# Autodesk Inventor assembly: SubAssembly
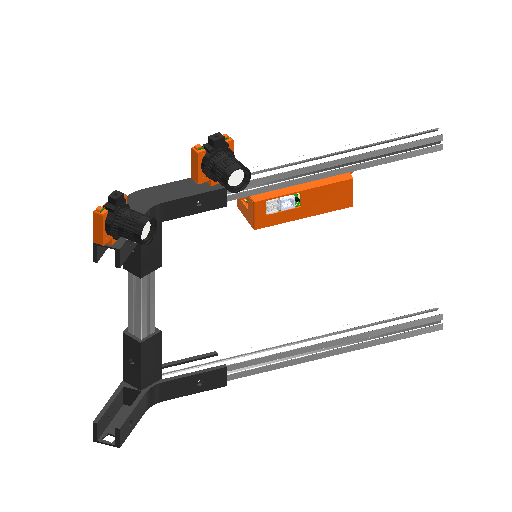
[picture p0: Inventor's stored thumbnail of the model, 512x512]
Saved by Autodesk Inventor 2025.2 (Build 292293000, 293)
## iProperties
Created: 2025-03-12
Part Number: SubAssembly
Document SubType Name: Assembly
Designer: rolan
Author: rolan
## Documents named in this file (6)
- C:\Users\rolan\Documents\PhD\Inventor\Assembly\SubAssembly.iam
- C:\Users\rolan\Documents\PhD\Inventor\Parts\135FootUpdate.ipt
- C:\Users\rolan\Documents\PhD\Inventor\Parts\Strut.ipt
- C:\Users\rolan\Documents\PhD\Inventor\Parts\Strut_short.ipt
- C:\Users\rolan\Documents\PhD\Inventor\Assembly\Camera.iam
- C:\Users\rolan\Documents\PhD\Inventor\Assembly\StereoPi.iam
## Components (8 placed, 5 different names)
1. 135FootUpdate:1 — Mate:1, Mate:2, Mate:3, Mate:26
2. Strut:1 — Mate:1, Mate:2, Mate:3
3. 135FootUpdate:2 — Mate:10, Mate:11, Mate:12, Mate:14, Mate:15, Flush:1, Mate:16, Mate:17, Mate:20, Mate:21, Mate:22, Mate:23, Mate:24, Mate:25
4. Strut:2 — Mate:10, Mate:11, Mate:12, Mate:13, Mate:18, Flush:20
5. Camera:1 [sub-assembly] — Mate:13, Mate:14, Mate:15, Mate:22, Mate:23
6. Camera:2 [sub-assembly] — Flush:1, Mate:16, Mate:17, Mate:20, Mate:21
7. StereoPi:1 [sub-assembly] — Mate:18, Flush:20
8. Strut_short:1 — Mate:24, Mate:25, Mate:26
## Relationships (21: Mate 19, Flush 2)
- Mate:1: 135FootUpdate:1 ↔ Strut:1
- Mate:2: 135FootUpdate:1 ↔ Strut:1
- Mate:3: 135FootUpdate:1 ↔ Strut:1
- Mate:10: 135FootUpdate:2 ↔ Strut:2
- Mate:11: 135FootUpdate:2 ↔ Strut:2
- Mate:12: 135FootUpdate:2 ↔ Strut:2
- Mate:13: Strut:2 ↔ Camera:1
- Mate:14: 135FootUpdate:2 ↔ Camera:1
- Mate:15: 135FootUpdate:2 ↔ Camera:1
- Flush:1: 135FootUpdate:2 ↔ Camera:2
- Mate:16: 135FootUpdate:2 ↔ Camera:2
- Mate:17: 135FootUpdate:2 ↔ Camera:2
- Mate:18: Strut:2 ↔ StereoPi:1
- Flush:20: Strut:2 ↔ StereoPi:1
- Mate:20: 135FootUpdate:2 ↔ Camera:2
- Mate:21: 135FootUpdate:2 ↔ Camera:2
- Mate:22: 135FootUpdate:2 ↔ Camera:1
- Mate:23: 135FootUpdate:2 ↔ Camera:1
- Mate:24: 135FootUpdate:2 ↔ Strut_short:1
- Mate:25: 135FootUpdate:2 ↔ Strut_short:1
- Mate:26: 135FootUpdate:1 ↔ Strut_short:1
